# Autodesk Inventor assembly: Барабан в сборке
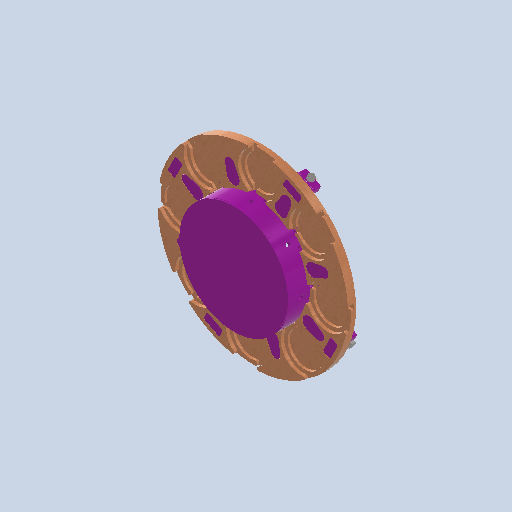
[picture p0: Inventor's stored thumbnail of the model, 512x512]
Saved by Autodesk Inventor 2024.1 (Build 281209000, 209)
## iProperties
Created: 2023-06-09
Part Number: Барабан в сборке
Document SubType Name: Assembly
Designer: Admin
Mass: 360.103 g
Surface Area: 2184.75 cm^2
Volume: 360.103 cm^3
Density: 1 g/cm^3
Author: Admin
## Documents named in this file (9)
- C:\Users\aleks\OneDrive\Рабочий стол\Хроматографический сортировщик\Детали\Барабан в сборке.iam
- C:\Users\aleks\OneDrive\Рабочий стол\Хроматографический сортировщик\Детали\Барабан.ipt
- C:\Users\aleks\OneDrive\Рабочий стол\Хроматографический сортировщик\Детали\Капсула.ipt
- C:\Users\aleks\OneDrive\Рабочий стол\Хроматографический сортировщик\Детали\Короб подшипника.ipt
- C:\Users\aleks\OneDrive\Рабочий стол\Хроматографический сортировщик\Детали\Покупные\Болт М5 15мм.ipt
- C:\Users\aleks\OneDrive\Рабочий стол\Хроматографический сортировщик\Детали\Покупные\Болт М5 10мм.ipt
- C:\Users\aleks\OneDrive\Рабочий стол\Хроматографический сортировщик\Детали\Покупные\Гайка М5 стопорная.ipt
- C:\Users\aleks\OneDrive\Рабочий стол\Хроматографический сортировщик\Детали\Покупные\Подшипник.ipt
- C:\Users\aleks\OneDrive\Рабочий стол\Хроматографический сортировщик\Детали\Покупные\Магнит.ipt
## Components (49 placed, 8 different names)
1. Барабан:1 — Совмещение:1, Заподлицо:1, Заподлицо:2, Заподлицо:3, Заподлицо:4, Совмещение:3, Совмещение:4, Совмещение:5, Совмещение:6, Совмещение:7, Совмещение:8, Совмещение:9, Совмещение:10, Совмещение:60, Совмещение:61, Совмещение:62, Совмещение:63, Совмещение:64, Совмещение:65, Совмещение:66, Совмещение:67, Совмещение:68, Совмещение:69, Совмещение:70, Совмещение:71, Совмещение:72, Совмещение:73, Совмещение:74, Совмещение:75, Совмещение:76, Совмещение:77, Совмещение:78, Совмещение:79, Совмещение:80, Совмещение:81, Совмещение:82, Совмещение:83, Совмещение:84
2. Капсула:1 — Совмещение:40, Заподлицо:7, Совмещение:51, Заподлицо:14, Угол:7, Совмещение:63, Совмещение:70, Совмещение:78
3. Капсула:2 — Совмещение:39, Заподлицо:10, Совмещение:45, Заподлицо:15, Угол:6, Совмещение:67, Совмещение:71, Совмещение:80
4. Капсула:3 — Совмещение:38, Заподлицо:11, Совмещение:46, Заподлицо:20, Угол:4, Совмещение:64, Совмещение:72, Совмещение:81
5. Капсула:4 — Совмещение:43, Заподлицо:6, Совмещение:50, Заподлицо:18, Угол:1, Совмещение:62, Совмещение:75, Совмещение:76
6. Капсула:5 — Совмещение:42, Заподлицо:9, Заподлицо:13, Совмещение:47, Заподлицо:17, Угол:8, Совмещение:66, Совмещение:74, Совмещение:83
7. Капсула:6 — Совмещение:41, Заподлицо:8, Совмещение:48, Заподлицо:16, Угол:3, Совмещение:61, Совмещение:69, Совмещение:77
8. Капсула:7 — Совмещение:37, Заподлицо:12, Совмещение:49, Заподлицо:19, Угол:5, Совмещение:65, Совмещение:73, Совмещение:82
9. Капсула:8 — Совмещение:36, Заподлицо:5, Совмещение:44, Заподлицо:21, Угол:2, Совмещение:60, Совмещение:68, Совмещение:79
10. Короб подшипника:1 — Заподлицо:3, Совмещение:5, Совмещение:6, Совмещение:13, Совмещение:17, Совмещение:22, Совмещение:27, Совмещение:33
11. Короб подшипника:2 — Заподлицо:4, Совмещение:7, Совмещение:8, Совмещение:12, Совмещение:18, Совмещение:20, Совмещение:23, Совмещение:30, Совмещение:31
12. Короб подшипника:3 — Заподлицо:2, Совмещение:9, Совмещение:10, Совмещение:14, Совмещение:15, Совмещение:21, Совмещение:29, Совмещение:34
13. Короб подшипника:4 — Заподлицо:1, Совмещение:3, Совмещение:4, Совмещение:11, Совмещение:16, Совмещение:19, Совмещение:28, Совмещение:32
14. Болт М5 15мм:1 — Совмещение:19, Совмещение:28
15. Болт М5 15мм:2 — Совмещение:20, Совмещение:30
16. Болт М5 15мм:3 — Совмещение:21, Совмещение:24, Совмещение:29
17. Болт М5 15мм:4 — Совмещение:22, Совмещение:26, Совмещение:27
18. Болт М5 10мм:1 — Совмещение:58, Заподлицо:26, Заподлицо:27
19. Болт М5 10мм:2 — Совмещение:55, Заподлицо:24, Заподлицо:25, Заподлицо:28
20. Болт М5 10мм:3 — Совмещение:54, Заподлицо:25, Заподлицо:26
21. Болт М5 10мм:4 — Совмещение:57, Заподлицо:22, Совмещение:84
22. Болт М5 10мм:5 — Совмещение:59, Заподлицо:27
23. Болт М5 10мм:6 — Совмещение:56, Заподлицо:23, Заподлицо:24
24. Болт М5 10мм:7 — Совмещение:53, Заподлицо:22, Заподлицо:23
25. Болт М5 10мм:8 — Совмещение:52, Заподлицо:28
26. Гайка М5 стопорная:1 — Совмещение:23, Совмещение:31
27. Гайка М5 стопорная:2 — Совмещение:24, Совмещение:34
28. Гайка М5 стопорная:3 — Совмещение:25, Совмещение:32
29. Гайка М5 стопорная:4 — Совмещение:26, Совмещение:33
30. Гайка М5 стопорная:5 — Совмещение:51, Заподлицо:14, Угол:7, Совмещение:53
31. Гайка М5 стопорная:6 — Совмещение:49, Заподлицо:19, Угол:5, Совмещение:55
32. Гайка М5 стопорная:7 — Совмещение:50, Заподлицо:18, Угол:1, Совмещение:58
33. Гайка М5 стопорная:8 — Совмещение:48, Заподлицо:16, Угол:3, Совмещение:57
34. Гайка М5 стопорная:9 — Совмещение:47, Заподлицо:17, Угол:8, Совмещение:52
35. Гайка М5 стопорная:10 — Совмещение:45, Заподлицо:15, Угол:6, Совмещение:54
36. Гайка М5 стопорная:11 — Совмещение:44, Заподлицо:21, Угол:2, Совмещение:59
37. Гайка М5 стопорная:12 — Совмещение:46, Заподлицо:20, Угол:4, Совмещение:56
38. Подшипник:1 — Совмещение:11, Совмещение:16, Совмещение:25
39. Подшипник:2 — Совмещение:12, Совмещение:18
40. Подшипник:3 — Совмещение:13, Совмещение:17
41. Подшипник:4 — Совмещение:14, Совмещение:15
42. Магнит:1 — Совмещение:36, Заподлицо:5
43. Магнит:2 — Совмещение:38, Заподлицо:11
44. Магнит:3 — Совмещение:41, Заподлицо:8
45. Магнит:4 — Совмещение:40, Заподлицо:7
46. Магнит:5 — Совмещение:43, Заподлицо:6
47. Магнит:6 — Совмещение:42, Заподлицо:9, Заподлицо:13
48. Магнит:7 — Совмещение:39, Заподлицо:10
49. Магнит:8 — Совмещение:37, Заподлицо:12
## Relationships (118: Mate 82, Flush 28, Angle 8)
- Совмещение:1 [Mate]: Барабан:1
- Заподлицо:1 [Flush]: Барабан:1 ↔ Короб подшипника:4
- Заподлицо:2 [Flush]: Барабан:1 ↔ Короб подшипника:3
- Заподлицо:3 [Flush]: Барабан:1 ↔ Короб подшипника:1
- Заподлицо:4 [Flush]: Барабан:1 ↔ Короб подшипника:2
- Совмещение:3 [Mate]: Барабан:1 ↔ Короб подшипника:4
- Совмещение:4 [Mate]: Барабан:1 ↔ Короб подшипника:4
- Совмещение:5 [Mate]: Барабан:1 ↔ Короб подшипника:1
- Совмещение:6 [Mate]: Барабан:1 ↔ Короб подшипника:1
- Совмещение:7 [Mate]: Барабан:1 ↔ Короб подшипника:2
- Совмещение:8 [Mate]: Барабан:1 ↔ Короб подшипника:2
- Совмещение:9 [Mate]: Барабан:1 ↔ Короб подшипника:3
- Совмещение:10 [Mate]: Барабан:1 ↔ Короб подшипника:3
- Совмещение:11 [Mate]: Короб подшипника:4 ↔ Подшипник:1
- Совмещение:12 [Mate]: Короб подшипника:2 ↔ Подшипник:2
- Совмещение:13 [Mate]: Короб подшипника:1 ↔ Подшипник:3
- Совмещение:14 [Mate]: Короб подшипника:3 ↔ Подшипник:4
- Совмещение:15 [Mate]: Короб подшипника:3 ↔ Подшипник:4
- Совмещение:16 [Mate]: Короб подшипника:4 ↔ Подшипник:1
- Совмещение:17 [Mate]: Короб подшипника:1 ↔ Подшипник:3
- Совмещение:18 [Mate]: Короб подшипника:2 ↔ Подшипник:2
- Совмещение:19 [Mate]: Короб подшипника:4 ↔ Болт М5 15мм:1
- Совмещение:20 [Mate]: Короб подшипника:2 ↔ Болт М5 15мм:2
- Совмещение:21 [Mate]: Короб подшипника:3 ↔ Болт М5 15мм:3
- Совмещение:22 [Mate]: Короб подшипника:1 ↔ Болт М5 15мм:4
- Совмещение:23 [Mate]: Короб подшипника:2 ↔ Гайка М5 стопорная:1
- Совмещение:24 [Mate]: Болт М5 15мм:3 ↔ Гайка М5 стопорная:2
- Совмещение:25 [Mate]: Гайка М5 стопорная:3 ↔ Подшипник:1
- Совмещение:26 [Mate]: Болт М5 15мм:4 ↔ Гайка М5 стопорная:4
- Совмещение:27 [Mate]: Короб подшипника:1 ↔ Болт М5 15мм:4
- Совмещение:28 [Mate]: Короб подшипника:4 ↔ Болт М5 15мм:1
- Совмещение:29 [Mate]: Короб подшипника:3 ↔ Болт М5 15мм:3
- Совмещение:30 [Mate]: Короб подшипника:2 ↔ Болт М5 15мм:2
- Совмещение:31 [Mate]: Короб подшипника:2 ↔ Гайка М5 стопорная:1
- Совмещение:32 [Mate]: Короб подшипника:4 ↔ Гайка М5 стопорная:3
- Совмещение:33 [Mate]: Короб подшипника:1 ↔ Гайка М5 стопорная:4
- Совмещение:34 [Mate]: Короб подшипника:3 ↔ Гайка М5 стопорная:2
- Совмещение:36 [Mate]: Капсула:8 ↔ Магнит:1
- Заподлицо:5 [Flush]: Капсула:8 ↔ Магнит:1
- Совмещение:37 [Mate]: Капсула:7 ↔ Магнит:8
- Совмещение:38 [Mate]: Капсула:3 ↔ Магнит:2
- Совмещение:39 [Mate]: Капсула:2 ↔ Магнит:7
- Совмещение:40 [Mate]: Капсула:1 ↔ Магнит:4
- Совмещение:41 [Mate]: Капсула:6 ↔ Магнит:3
- Совмещение:42 [Mate]: Капсула:5 ↔ Магнит:6
- Совмещение:43 [Mate]: Капсула:4 ↔ Магнит:5
- Заподлицо:6 [Flush]: Капсула:4 ↔ Магнит:5
- Заподлицо:7 [Flush]: Капсула:1 ↔ Магнит:4
- Заподлицо:8 [Flush]: Капсула:6 ↔ Магнит:3
- Заподлицо:9 [Flush]: Капсула:5 ↔ Магнит:6
- Заподлицо:10 [Flush]: Капсула:2 ↔ Магнит:7
- Заподлицо:11 [Flush]: Капсула:3 ↔ Магнит:2
- Заподлицо:12 [Flush]: Капсула:7 ↔ Магнит:8
- Заподлицо:13 [Flush]: Капсула:5 ↔ Магнит:6
- Совмещение:44 [Mate]: Капсула:8 ↔ Гайка М5 стопорная:11
- Совмещение:45 [Mate]: Капсула:2 ↔ Гайка М5 стопорная:10
- Совмещение:46 [Mate]: Капсула:3 ↔ Гайка М5 стопорная:12
- Совмещение:47 [Mate]: Капсула:5 ↔ Гайка М5 стопорная:9
- Совмещение:48 [Mate]: Капсула:6 ↔ Гайка М5 стопорная:8
- Совмещение:49 [Mate]: Капсула:7 ↔ Гайка М5 стопорная:6
- Совмещение:50 [Mate]: Капсула:4 ↔ Гайка М5 стопорная:7
- Совмещение:51 [Mate]: Капсула:1 ↔ Гайка М5 стопорная:5
- Заподлицо:14 [Flush]: Капсула:1 ↔ Гайка М5 стопорная:5
- Заподлицо:15 [Flush]: Капсула:2 ↔ Гайка М5 стопорная:10
- Заподлицо:16 [Flush]: Капсула:6 ↔ Гайка М5 стопорная:8
- Заподлицо:17 [Flush]: Капсула:5 ↔ Гайка М5 стопорная:9
- Заподлицо:18 [Flush]: Капсула:4 ↔ Гайка М5 стопорная:7
- Заподлицо:19 [Flush]: Капсула:7 ↔ Гайка М5 стопорная:6
- Заподлицо:20 [Flush]: Капсула:3 ↔ Гайка М5 стопорная:12
- Заподлицо:21 [Flush]: Капсула:8 ↔ Гайка М5 стопорная:11
- Угол:1 [Angle] (0 deg): Капсула:4 ↔ Гайка М5 стопорная:7
- Угол:2 [Angle] (0 deg): Капсула:8 ↔ Гайка М5 стопорная:11
- Угол:3 [Angle] (0 deg): Капсула:6 ↔ Гайка М5 стопорная:8
- Угол:4 [Angle] (0 deg): Капсула:3 ↔ Гайка М5 стопорная:12
- Угол:5 [Angle] (0 deg): Капсула:7 ↔ Гайка М5 стопорная:6
- Угол:6 [Angle] (0 deg): Капсула:2 ↔ Гайка М5 стопорная:10
- Угол:7 [Angle] (0 deg): Капсула:1 ↔ Гайка М5 стопорная:5
- Угол:8 [Angle] (0 deg): Капсула:5 ↔ Гайка М5 стопорная:9
- Совмещение:52 [Mate]: Болт М5 10мм:8 ↔ Гайка М5 стопорная:9
- Совмещение:53 [Mate]: Болт М5 10мм:7 ↔ Гайка М5 стопорная:5
- Совмещение:54 [Mate]: Болт М5 10мм:3 ↔ Гайка М5 стопорная:10
- Совмещение:55 [Mate]: Болт М5 10мм:2 ↔ Гайка М5 стопорная:6
- Совмещение:56 [Mate]: Болт М5 10мм:6 ↔ Гайка М5 стопорная:12
- Совмещение:57 [Mate]: Болт М5 10мм:4 ↔ Гайка М5 стопорная:8
- Совмещение:58 [Mate]: Болт М5 10мм:1 ↔ Гайка М5 стопорная:7
- Совмещение:59 [Mate]: Болт М5 10мм:5 ↔ Гайка М5 стопорная:11
- Совмещение:60 [Mate]: Барабан:1 ↔ Капсула:8
- Совмещение:61 [Mate]: Барабан:1 ↔ Капсула:6
- Совмещение:62 [Mate]: Барабан:1 ↔ Капсула:4
- Совмещение:63 [Mate]: Барабан:1 ↔ Капсула:1
- Совмещение:64 [Mate]: Барабан:1 ↔ Капсула:3
- Совмещение:65 [Mate]: Барабан:1 ↔ Капсула:7
- Совмещение:66 [Mate]: Барабан:1 ↔ Капсула:5
- Совмещение:67 [Mate]: Барабан:1 ↔ Капсула:2
- Совмещение:68 [Mate]: Барабан:1 ↔ Капсула:8
- Совмещение:69 [Mate]: Барабан:1 ↔ Капсула:6
- Совмещение:70 [Mate]: Барабан:1 ↔ Капсула:1
- Совмещение:71 [Mate]: Барабан:1 ↔ Капсула:2
- Совмещение:72 [Mate]: Барабан:1 ↔ Капсула:3
- Совмещение:73 [Mate]: Барабан:1 ↔ Капсула:7
- Совмещение:74 [Mate]: Барабан:1 ↔ Капсула:5
- Совмещение:75 [Mate]: Барабан:1 ↔ Капсула:4
- Совмещение:76 [Mate]: Барабан:1 ↔ Капсула:4
- Совмещение:77 [Mate]: Барабан:1 ↔ Капсула:6
- Совмещение:78 [Mate]: Барабан:1 ↔ Капсула:1
- Совмещение:79 [Mate]: Барабан:1 ↔ Капсула:8
- Совмещение:80 [Mate]: Барабан:1 ↔ Капсула:2
- Совмещение:81 [Mate]: Барабан:1 ↔ Капсула:3
- Совмещение:82 [Mate]: Барабан:1 ↔ Капсула:7
- Совмещение:83 [Mate]: Барабан:1 ↔ Капсула:5
- Заподлицо:22 [Flush]: Болт М5 10мм:4 ↔ Болт М5 10мм:7
- Заподлицо:23 [Flush]: Болт М5 10мм:6 ↔ Болт М5 10мм:7
- Заподлицо:24 [Flush]: Болт М5 10мм:2 ↔ Болт М5 10мм:6
- Заподлицо:25 [Flush]: Болт М5 10мм:2 ↔ Болт М5 10мм:3
- Заподлицо:26 [Flush]: Болт М5 10мм:1 ↔ Болт М5 10мм:3
- Заподлицо:27 [Flush]: Болт М5 10мм:1 ↔ Болт М5 10мм:5
- Заподлицо:28 [Flush]: Болт М5 10мм:2 ↔ Болт М5 10мм:8
- Совмещение:84 [Mate]: Барабан:1 ↔ Болт М5 10мм:4
